# Autodesk Inventor assembly: Drive Roller Assembly 2
(part 2 of 2)
- Mate:983: Vex Pro 1x1 rectangular tubing 14 in length:5 ↔ Bearing Mount Spacer 1-8 in:5
- Mate:984: Roller Piston 4 (.5 and 1 in Stroke, 9-16 in Bore):1 ↔ Shaft Collar 3-16 in ID (6435K510):2
- Mate:985: Roller Piston 4 (.5 and 1 in Stroke, 9-16 in Bore):1 ↔ Shaft Collar 3-16 in ID (6435K510):1
- Mate:986: Bracket:1 ↔ Roller Piston 4 (.5 and 1 in Stroke, 9-16 in Bore):2
- Mate:987: Roller Piston 4 (.5 and 1 in Stroke, 9-16 in Bore):2 ↔ Shaft Collar 3-16 in ID (6435K510):3
- Mate:988: Vex Pro 1x1 rectangular tubing 14 in length (roller):1 ↔ Side Mount Custom:1
- Mate:989: Vex Pro 1x1 rectangular tubing 14 in length (roller):1 ↔ Side Mount Custom:1
- Mate:990: VersaPlanetary (Fixed):1 ↔ Side Mount Custom:1
- Mate:991: VersaPlanetary (Fixed):1 ↔ Side Mount Custom:1
- Mate:992: VersaPlanetary (Fixed):1 ↔ Side Mount Custom:1
## Named parameters: d216_d210 = 0 mm, d217_d213 = 0 mm, d240_d195 = 0 mm, d241_d196 = 0 mm, d242_d197 = 0 mm, d243_d198 = 0 mm, d305_d302 = 0 mm, d306_d303 = 0 mm, d307_d304 = 0 mm, d334_d317 = 0 mm, d335_d318 = -19.05 mm, d336_d325 = 0 mm, d339_d304 = 0 mm, d343_d308 = 0 mm, d344_d309 = 0 mm, d345_d310 = 0 mm, d346_d316 = 0 mm, d347_d326 = 0 mm, d348_d327 = -7.14375 mm, d349_d328 = 0 mm, d350_d329 = 0 mm, d351_d330 = 0 mm, d352_d331 = 0 mm, d353_d332 = 0 mm, d354_d333 = 0 mm, d770_d743 = 0 mm, d771_d744 = 0 mm, d772_d745 = 0 mm, d773_d746 = 0 mm, d774_d750 = 2.38125 mm, d791_d742 = 0 mm
